# Autodesk Inventor assembly: A_Trockenzelle
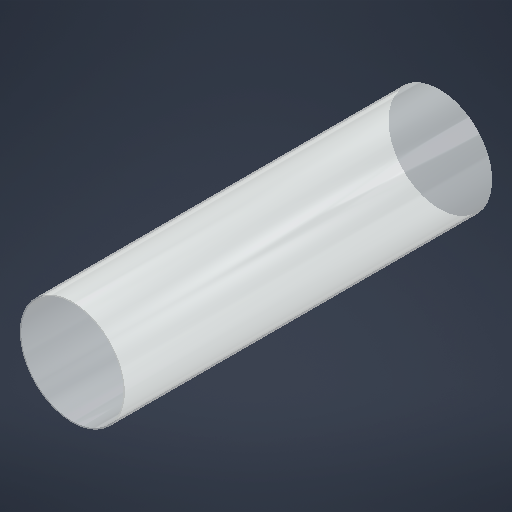
[picture p0: Inventor's stored thumbnail of the model, 512x512]
Saved by Autodesk Inventor 2026 (Build 300175000, 175)
## iProperties
Created: 2025-04-26
Part Number: A_Trockenzelle
Document SubType Name: Assembly
Designer: FAL
Author: FAL
## Documents named in this file (2)
- C:\Users\FAL\Desktop\git\U-BERT\CAD\Trockenzelle\A_Trockenzelle.iam
- C:\Users\FAL\Desktop\git\U-BERT\CAD\Trockenzelle\P_Kunststoffrohr.ipt
## Components (1 placed, 1 different names)
1. P_Kunststoffrohr:1 — Fluchtend:1, Fluchtend:2, Fluchtend:3
## Relationships (3: Flush 3)
- Fluchtend:1 [Flush]: P_Kunststoffrohr:1
- Fluchtend:2 [Flush]: P_Kunststoffrohr:1
- Fluchtend:3 [Flush]: P_Kunststoffrohr:1
